# Autodesk Inventor assembly: am14u3LongWithArmAndGripper
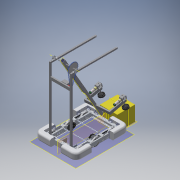
[picture p0: Inventor's stored thumbnail of the model, 180x180]
Saved by Autodesk Inventor 2018.2 (Build 222227000, 227)
## iProperties
Created: 2018-01-15
Part Number: am14u3LongWithArmAndGripper
Document SubType Name: Assembly
Designer: steele
Author: steele
## Documents named in this file (5)
- D:\snobotics\CAD-Development\robSteele\2018-FRC\am14u3LongWithArmAndGripper.iam
- D:\snobotics\CAD-Development\robSteele\2018-FRC\AMbaseLongWithBumper\Long with Bumper\DB_DriveBaseLong_AM14U3_Bumpers and Battery Tray.iam
- D:\snobotics\CAD-Development\robSteele\2018-FRC\Field Elements\Cube-GE-18124.ipt
- D:\snobotics\CAD-Development\robSteele\2018-FRC\Gripper\gripperAssembly.iam
- D:\snobotics\CAD-Development\robSteele\2018-FRC\Arm\ArmFrameWithMotorAndGears.iam
## Components (4 placed, 4 different names)
1. DB_DriveBaseLong_AM14U3_Bumpers and Battery Tray:1 [sub-assembly] — Flush:2, Mate:7, Mate:8, Mate:9, Mate:10
2. Cube-GE-18124:1
3. gripperAssembly:1 [sub-assembly] — Mate:7
4. ArmFrameWithMotorAndGears:1 [sub-assembly] — Mate:8, Mate:9, Mate:10
## Relationships (5: Mate 4, Flush 1)
- Flush:2 (50.8 mm): DB_DriveBaseLong_AM14U3_Bumpers and Battery Tray:1
- Mate:7: DB_DriveBaseLong_AM14U3_Bumpers and Battery Tray:1 ↔ gripperAssembly:1
- Mate:8: DB_DriveBaseLong_AM14U3_Bumpers and Battery Tray:1 ↔ ArmFrameWithMotorAndGears:1
- Mate:9: DB_DriveBaseLong_AM14U3_Bumpers and Battery Tray:1 ↔ ArmFrameWithMotorAndGears:1
- Mate:10: DB_DriveBaseLong_AM14U3_Bumpers and Battery Tray:1 ↔ ArmFrameWithMotorAndGears:1
